# Autodesk Inventor assembly: juzzruchem
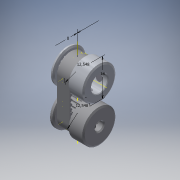
[picture p0: Inventor's stored thumbnail of the model, 180x180]
Saved by Autodesk Inventor 2019 (Build 230136000, 136)
## iProperties
Created: 2020-05-17
Part Number: juzzruchem
Document SubType Name: Assembly
Designer: estee
Author: estee
## Documents named in this file (6)
- C:\Users\estee\OneDrive\Pulpit\estere\1\MUM\projejt\juzzruchem.iam
- C:\Users\estee\OneDrive\Pulpit\estere\1\MUM\projejt\przekladnia.ipt
- C:\Users\estee\OneDrive\Pulpit\estere\1\MUM\projejt\zab.ipt
- C:\Users\estee\OneDrive\Pulpit\estere\1\MUM\projejt\pasek.ipt
- C:\Users\estee\OneDrive\Pulpit\estere\1\MUM\projejt\kolooooo.ipt
- C:\Users\estee\OneDrive\Pulpit\estere\1\MUM\projejt\kolo2\GT2_20T-sh8.ipt
## Components (42 placed, 5 different names)
1. przekladnia:1 — Flush:1, Flush:2, Flush:3, Drive-1, Angle:1, Mate:2, Angle:2, Mate:3, Mate:4, Mate:5, Mate:7, Mate:9
2. pasek:1 — Mate:3, Mate:4, Mate:5
3. kolooooo:1 — Mate:6, Mate:7, Rotation:1, Drive-2
4. GT2_20T-sh8:1 — Mate:8, Mate:9, Rotation:1
5. zab:1 — Drive-1, Flush:4, Angle:1
6. zab:2
7. zab:3
8. zab:4
9. zab:5
10. zab:6
11. zab:7
12. zab:8
13. zab:9
14. zab:10
15. zab:11
16. zab:12
17. zab:13
18. zab:14
19. zab:15
20. zab:16
21. zab:17
22. zab:18
23. zab:19
24. zab:20
25. zab:21
26. zab:22
27. zab:23
28. zab:24
29. zab:25
30. zab:26
31. zab:27
32. zab:28
33. zab:29
34. zab:30
35. zab:31
36. zab:32
37. zab:33
38. zab:34
39. zab:35
40. zab:36
41. zab:37
42. zab:38
## Component patterns: (38 elements, first: zab:1)
## Relationships (17: Mate 9, Flush 4, Angle 3, RelateRotation 1)
- Flush:1: przekladnia:1
- Flush:2: przekladnia:1
- Flush:3: przekladnia:1
- Drive-1 [Mate]: przekladnia:1 ↔ zab:1
- Flush:4 (-3 mm): zab:1
- Angle:1 (0 deg): przekladnia:1 ↔ zab:1
- Mate:2: przekladnia:1
- Angle:2 (0 deg): przekladnia:1
- Mate:3: przekladnia:1 ↔ pasek:1
- Mate:4: przekladnia:1 ↔ pasek:1
- Mate:5 (3 mm): przekladnia:1 ↔ pasek:1
- Mate:6: kolooooo:1
- Mate:7 (10.95 mm): przekladnia:1 ↔ kolooooo:1
- Mate:8: GT2_20T-sh8:1
- Mate:9 (10.95 mm): przekladnia:1 ↔ GT2_20T-sh8:1
- Rotation:1 [RelateRotation] (1 ul): kolooooo:1 ↔ GT2_20T-sh8:1
- Drive-2 [Angle] (0 deg): kolooooo:1
